# Autodesk Inventor assembly: SubSistemaLiberacion
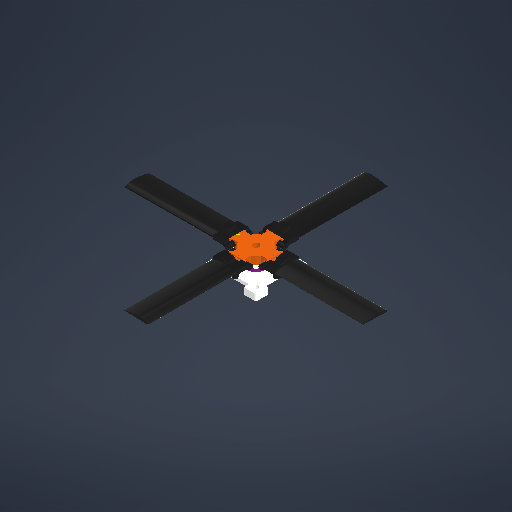
[picture p0: Inventor's stored thumbnail of the model, 512x512]
Saved by Autodesk Inventor 2026.1 (Build 301233000, 233)
## iProperties
Created: 2025-12-08
Part Number: SubSistemaLiberacion
Document SubType Name: Assembly
Designer: vickh
Author: vickh
## Documents named in this file (7)
- C:\Users\vickh\Documents\Proyectos\Cansat_Huitzilin\3D\NuevoDiseno\SubSistemaLiberacion.iam
- C:\Users\vickh\Documents\Proyectos\Cansat_Huitzilin\3D\NuevoDiseno\SujeccionHelices.ipt
- C:\Users\vickh\Documents\Proyectos\Cansat_Huitzilin\3D\NuevoDiseno\expansor de conexion.ipt
- C:\Users\vickh\Downloads\Bearing 625 2RS\Bearing 625 2RS\Bearing 625 2RS.ipt
- C:\Users\vickh\Documents\Proyectos\Cansat_Huitzilin\3D\NuevoDiseno\Pala.ipt
- C:\Users\vickh\Documents\Proyectos\Cansat_Huitzilin\3D\NuevoDiseno\SistemaLiberacion2.2.ipt
- C:\Users\vickh\Documents\Proyectos\Cansat_Huitzilin\3D\NuevoDiseno\SistemLiberacion1.ipt
## Components (9 placed, 6 different names)
1. SujeccionHelices:1 — Insertar:1, De rotación:1, De rotación:2, De rotación:3, De rotación:4
2. expansor de conexion:1 — Insertar:2, Insertar:3
3. Bearing 625 2RS:1 — Insertar:1, Insertar:2
4. Pala:1 — De rotación:1
5. Pala:2 — De rotación:3
6. Pala:3 — De rotación:4
7. Pala:4 — De rotación:2
8. SistemaLiberacion2.2:1 — Insertar:3, Cilíndrica:1
9. SistemLiberacion1:1 — Cilíndrica:1
## Relationships (8: RevoluteJoint 4, Insert 3, CylindricalJoint 1)
- Insertar:1: SujeccionHelices:1 ↔ Bearing 625 2RS:1
- Insertar:2: expansor de conexion:1 ↔ Bearing 625 2RS:1
- De rotación:1 [RevoluteJoint]: SujeccionHelices:1 ↔ Pala:1
- De rotación:2 [RevoluteJoint]: SujeccionHelices:1 ↔ Pala:4
- De rotación:3 [RevoluteJoint]: SujeccionHelices:1 ↔ Pala:2
- De rotación:4 [RevoluteJoint]: SujeccionHelices:1 ↔ Pala:3
- Insertar:3 (0.1 mm): expansor de conexion:1 ↔ SistemaLiberacion2.2:1
- Cilíndrica:1 [CylindricalJoint]: SistemaLiberacion2.2:1 ↔ SistemLiberacion1:1
